# Autodesk Inventor assembly: Flange_tube_MIR1
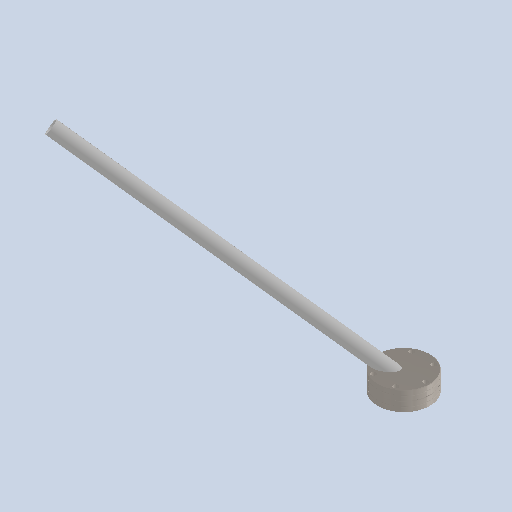
[picture p0: Inventor's stored thumbnail of the model, 512x512]
Saved by Autodesk Inventor 2024 (Build 280153000, 153)
## iProperties
Created: 2024-11-06
Part Number: Flange_tube_MIR1
Document SubType Name: Assembly
Designer: Andreas Weber
Author: Andreas Weber
## Documents named in this file (4)
- C:\Users\Andreas Weber\Desktop\Upload for Github\Flange_tube_MIR1.iam
- C:\Users\Andreas Weber\Desktop\Upload for Github\blank_flange_CF40_MIR1.ipt
- C:\Users\Andreas Weber\Desktop\Upload for Github\blank_flange_thread_CF40_MIR1.ipt
- C:\Users\Andreas Weber\Desktop\Upload for Github\tube_Brewster_angle_MIR1.ipt
## Components (3 placed, 3 different names)
1. blank_flange_CF40_MIR1:1 — Drehbar:1, Verschiebbar:1
2. blank_flange_thread_CF40_MIR1:1 — Drehbar:1
3. tube_Brewster_angle_MIR1:1 — Verschiebbar:1
## Relationships (2: RevoluteJoint 1, TranslationJoint 1)
- Drehbar:1 [RevoluteJoint]: blank_flange_CF40_MIR1:1 ↔ blank_flange_thread_CF40_MIR1:1
- Verschiebbar:1 [TranslationJoint]: blank_flange_CF40_MIR1:1 ↔ tube_Brewster_angle_MIR1:1
